# Autodesk Inventor assembly: NRF24L01L+Antenna
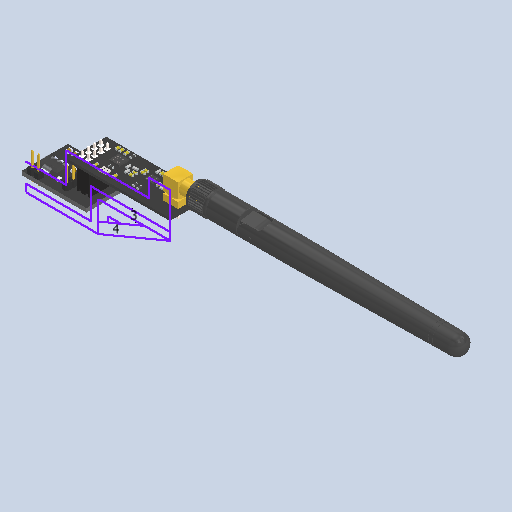
[picture p0: Inventor's stored thumbnail of the model, 512x512]
Saved by Autodesk Inventor 2024 (Build 280153000, 153)
## iProperties
Created: 2019-01-18
Part Number: NRF24L01L+Antenna
Document SubType Name: Assembly
Designer: 18179
Sending System: SolidWorks 2016
Last Author: Condor
Last Saved: 2019-01-20
Author: 18179
## Documents named in this file (4)
- C:\Users\18179\Desktop\TuppyMkIV_GitHub\TuppyMkIV\CAD\NRF24L01L+Antenna\NRF24L01L+Antenna.iam
- C:\Users\18179\Desktop\TuppyMkIV_GitHub\TuppyMkIV\CAD\NRF24L01L+Antenna\NRF24L01L.ipt
- C:\Users\18179\Desktop\TuppyMkIV_GitHub\TuppyMkIV\CAD\NRF24L01L+Antenna\Antenna assy.iam
- C:\Users\18179\Downloads\nrf24l01-power-adapter-1.snapshot.19\NRFL24L01_Power_Board_asm\NRFL24L01_Power_Board_asm.iam
## Components (3 placed, 3 different names)
1. NRF24L01L:1 — Mate:1, Mate:2, Mate:3, Mate:4, Mate:5
2. Antenna assy:1 [sub-assembly] — Mate:4, Mate:5
3. NRFL24L01_Power_Board_asm:1 [sub-assembly] — Mate:1, Mate:2, Mate:3
## Relationships (5: Mate 5)
- Mate:1: NRF24L01L:1 ↔ NRFL24L01_Power_Board_asm:1
- Mate:2: NRF24L01L:1 ↔ NRFL24L01_Power_Board_asm:1
- Mate:3: NRF24L01L:1 ↔ NRFL24L01_Power_Board_asm:1
- Mate:4: NRF24L01L:1 ↔ Antenna assy:1
- Mate:5: NRF24L01L:1 ↔ Antenna assy:1
